# Autodesk Inventor assembly: Assembly_Dedo
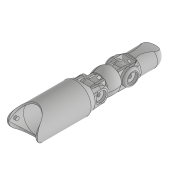
[picture p0: Inventor's stored thumbnail of the model, 180x180]
Saved by Autodesk Inventor 2020 (Build 240168000, 168)
## iProperties
Created: 2021-03-24
Part Number: Assembly_Dedo
Document SubType Name: Assembly
Designer: deox
Author: deox
## Documents named in this file (7)
- C:\Users\deox\Desktop\TCC\Inventor Files\Dedo Kick\Assembly_Dedo.iam
- C:\Users\deox\Desktop\TCC\Inventor Files\Dedo Kick\Base.ipt
- C:\Users\deox\Desktop\TCC\Inventor Files\Dedo Kick\Middle.ipt
- C:\Users\deox\Desktop\TCC\Inventor Files\Dedo Kick\ShameHider.ipt
- C:\Users\deox\Desktop\TCC\Inventor Files\Dedo Kick\Tip.ipt
- C:\Users\deox\Desktop\TCC\Inventor Files\Dedo Kick\TipTip.ipt
- C:\Users\deox\Desktop\TCC\Inventor Files\Dedo Kick\Socket.ipt
## Components (6 placed, 6 different names)
1. Base:1 — Mate:1, Mate:2, Mate:10, Mate:11, Angle:1
2. Middle:1 — Mate:1, Mate:2, Mate:3, Mate:4, Mate:5, Mate:6, Mate:7
3. ShameHider:1 — Mate:3, Mate:4, Mate:5
4. Tip:1 — Mate:6, Mate:7, Mate:8, Mate:9
5. TipTip:1 — Mate:8, Mate:9
6. Socket:1 — Mate:10, Mate:11, Angle:1
## Relationships (12: Mate 11, Angle 1)
- Mate:1: Base:1 ↔ Middle:1
- Mate:2: Base:1 ↔ Middle:1
- Mate:3: Middle:1 ↔ ShameHider:1
- Mate:4: Middle:1 ↔ ShameHider:1
- Mate:5: Middle:1 ↔ ShameHider:1
- Mate:6: Middle:1 ↔ Tip:1
- Mate:7: Middle:1 ↔ Tip:1
- Mate:8: Tip:1 ↔ TipTip:1
- Mate:9: Tip:1 ↔ TipTip:1
- Mate:10: Base:1 ↔ Socket:1
- Mate:11: Base:1 ↔ Socket:1
- Angle:1 (0 deg): Base:1 ↔ Socket:1
